# Autodesk Inventor assembly: Openbuilds_Dual_V-Wheel
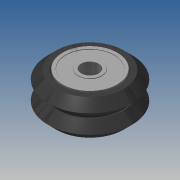
[picture p0: Inventor's stored thumbnail of the model, 180x180]
Saved by Autodesk Inventor 2015 (Build 190159000, 159)
## iProperties
Created: 2015-01-09
Part Number: Openbuilds_Dual_V-Wheel
Document SubType Name: Assembly
Designer: Marc
Author: Marc
## Documents named in this file (4)
- E:\Modellflieger\3D Drucker\MotediusQR 500mm\Openbuilds_Dual_V-Wheel\Openbuilds_Dual_V-Wheel.iam
- E:\Modellflieger\3D Drucker\MotediusQR 500mm\Openbuilds_Dual_V-Wheel\Delrin_Dual_V.ipt
- E:\Modellflieger\3D Drucker\MotediusQR 500mm\Openbuilds_Dual_V-Wheel\Kugellager625_5x16x5.ipt
- C:\Users\Marc\Documents\Inventor\Content Center Files\R2015\de-DE\DIN 125-1  A\DIN 125 - A 5,3.ipt
## Components (4 placed, 3 different names)
1. Delrin_Dual_V:1 — Einfügen:1, Einfügen:2, Einfügen:3
2. Kugellager625_5x16x5:1 — Einfügen:1
3. Kugellager625_5x16x5:2 — Einfügen:3
4. DIN 125-1 A A 5,3:1 — Einfügen:2
## Relationships (3: Insert 3)
- Einfügen:1 [Insert]: Delrin_Dual_V:1 ↔ Kugellager625_5x16x5:1
- Einfügen:2 [Insert]: Delrin_Dual_V:1 ↔ DIN 125-1 A A 5,3:1
- Einfügen:3 [Insert]: Delrin_Dual_V:1 ↔ Kugellager625_5x16x5:2
